# Autodesk Inventor assembly: Leg_joint_roll_pitch
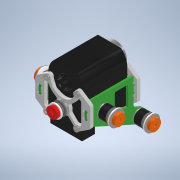
[picture p0: Inventor's stored thumbnail of the model, 180x180]
Saved by Autodesk Inventor 2020 (Build 240168000, 168)
## iProperties
Part Number: Leg_joint_roll_pitch
Document SubType Name: Assembly
Designer: Masato Kubotera
Mass: 101.309 g
Surface Area: 368.925 cm^2
Volume: 74.117 cm^3
Density: 1.36688 g/cm^3
Author: Masato Kubotera
## Documents named in this file (20)
- C:\Users\MasatoKubotera\Documents\Inventor\SUSTAINA-OP\LowerBody\Leg_joit\Leg_joint_roll_pitch.iam
- C:\Users\MasatoKubotera\Documents\Inventor\SUSTAINA-OP\LowerBody\Leg_joit\Leg_joint_pitch_frame.ipt
- C:\Users\MasatoKubotera\Documents\Inventor\SUSTAINA-OP\LowerBody\Leg_joit\Leg_joint_roll_frame.ipt
- C:\Users\MasatoKubotera\Documents\Inventor\SUSTAINA-OP\ReadyMade\Screw\M2_6-20.ipt
- C:\Users\MasatoKubotera\Documents\Inventor\SUSTAINA-OP\ReadyMade\Screw\M2_6-15.ipt
- C:\Users\MasatoKubotera\Documents\Inventor\SUSTAINA-OP\ReadyMade\Bush\80F-0603.ipt
- C:\Users\MasatoKubotera\Documents\Inventor\SUSTAINA-OP\ReadyMade\Washer\CC-0612-50B.ipt
- C:\Users\MasatoKubotera\Documents\Inventor\SUSTAINA-OP\ReadyMade\InsertNut\SF419.ipt
- C:\Users\MasatoKubotera\Documents\Inventor\SUSTAINA-OP\ReadyMade\Washer\UUW-0412-10H.ipt
- C:\Users\MasatoKubotera\Documents\Inventor\SUSTAINA-OP\ReadyMade\Spacer\SLSBF6-39.5-M4-N4.ipt
- C:\Users\MasatoKubotera\Documents\Inventor\SUSTAINA-OP\ReadyMade\Screw\DBTS4-11-6-DHC.ipt
- C:\Users\MasatoKubotera\Documents\Inventor\SUSTAINA-OP\ReadyMade\Screw\DBTS4-5-5-DHC.ipt
- C:\Users\MasatoKubotera\Documents\Inventor\SUSTAINA-OP\ReadyMade\Screw\DBTS4-10-4-DHC.ipt
- C:\Users\MasatoKubotera\Documents\Inventor\SUSTAINA-OP\ReadyMade\InsertNut\S4-05-3W.ipt
- C:\Users\MasatoKubotera\Documents\Inventor\SUSTAINA-OP\ReadyMade\Screw\DBTS4-11-8-DHC.ipt
- C:\Users\MasatoKubotera\Documents\Inventor\SUSTAINA-OP\ReadyMade\Washer\UUW-0614-05H.ipt
- C:\Users\MasatoKubotera\Documents\Inventor\SUSTAINA-OP\ReadyMade\Washer\TT-0612-10.ipt
- C:\Users\MasatoKubotera\Documents\Inventor\SUSTAINA-OP\ReadyMade\Washer\TT-0814-10.ipt
- C:\Users\MasatoKubotera\Documents\Inventor\SUSTAINA-OP\ReadyMade\Washer\CCC-0612-65B.ipt
- C:\Users\MasatoKubotera\Documents\Inventor\SUSTAINA-OP\ReadyMade\KONDO\B3M-SC-1170-A_with_ClampHorn.iam
## Components (50 placed, 19 different names)
1. Leg_joint_roll_frame:1 — 挿入:5, 挿入:6, 挿入:7, 挿入:8, 挿入:9, 挿入:10, 角度:1, フラッシュ:2, メイト:3, メイト:4, メイト:5, 挿入:248, 挿入:249
2. Leg_joint_roll_frame:2 — 挿入:15, 挿入:16, 挿入:17, 挿入:18, 角度:2, 角度:4, 挿入:246, 挿入:247
3. Leg_joint_pitch_frame:1 — フラッシュ:3, 挿入:19, フラッシュ:4, メイト:5, 挿入:20, 挿入:21, 挿入:22
4. Leg_joint_pitch_frame:2 — フラッシュ:2, フラッシュ:3, フラッシュ:4, メイト:3, メイト:4, 挿入:23, 挿入:24, 挿入:25, 挿入:26
5. 80F-0603:1 — 挿入:43
6. 80F-0603:2 — 挿入:44
7. 80F-0603:3 — 挿入:243
8. 80F-0603:4 — 挿入:242
9. 80F-0603:5 — 挿入:244
10. 80F-0603:6 — 挿入:245
11. UUW-0412-10BH:1 — 挿入:9, 挿入:27
12. UUW-0412-10BH:2 — 挿入:17, 挿入:28, 挿入:33
13. UUW-0412-10BH:3 — 挿入:19, 挿入:226, 挿入:241
14. UUW-0412-10BH:4 — 挿入:22, 挿入:35, 挿入:240
15. UUW-0412-10BH:5 — 挿入:23, 挿入:227, 挿入:239
16. UUW-0412-10BH:6 — 挿入:26, 挿入:37, 挿入:238
17. UUW-0412-10BH:7 — 挿入:27, 挿入:38, 挿入:43
18. CC-0612-50B:5 — 挿入:28, 挿入:44
19. SF419:1 — 挿入:25
20. SF419:2 — 挿入:20
21. S4-05-3W:1 — 挿入:10, 角度:1
22. S4-05-3W:2 — 挿入:18, 角度:2
23. SLSBF6-39.5-M4-N4:1 — 挿入:21, 挿入:24, 角度:4
24. DBS4-5-5:1 — 挿入:38, 挿入:232
25. DBTS4-11-6:3 — 挿入:37, 挿入:229
26. DBTS4-11-6:4 — 挿入:35, 挿入:230
27. DBTS4-10-4:1 — 挿入:33, 挿入:233
28. DBTS4-11-8:1 — 挿入:226, 挿入:231
29. DBTS4-11-8:2 — 挿入:227, 挿入:228
30. UUW-0614-05BH:1 — 挿入:228, 挿入:234
31. UUW-0614-05BH:2 — 挿入:229, 挿入:235
32. UUW-0614-05BH:3 — 挿入:230, 挿入:236
33. UUW-0614-05BH:4 — 挿入:231, 挿入:237
34. TT-0612-10:1 — 挿入:233
35. TT-0612-10:2 — 挿入:232
36. TT-0814-10:1 — 挿入:234
37. TT-0814-10:2 — 挿入:235
38. TT-0814-10:3 — 挿入:237
39. TT-0814-10:4 — 挿入:236
40. CCC-0612-65B:1 — 挿入:238, 挿入:245
41. CCC-0612-65B:2 — 挿入:241, 挿入:243
42. CCC-0612-65B:3 — 挿入:239, 挿入:244
43. CCC-0612-65B:4 — 挿入:240, 挿入:242
44. B3M-SC-1170-A_with_ClampHorn:1 [sub-assembly] — 挿入:246, 挿入:247, 挿入:248, 挿入:249
45. M2_6-20:1 — 挿入:7
46. M2_6-20:2 — 挿入:8
47. M2_6-20:3 — 挿入:5
48. M2_6-20:4 — 挿入:6
49. M2_6-15:2 — 挿入:16
50. M2_6-15:3 — 挿入:15
## Relationships (59: Insert 50, Angle 3, Flush 3, Mate 3)
- 挿入:5 [Insert]: Leg_joint_roll_frame:1 ↔ M2_6-20:3
- 挿入:6 [Insert]: Leg_joint_roll_frame:1 ↔ M2_6-20:4
- 挿入:7 [Insert]: Leg_joint_roll_frame:1 ↔ M2_6-20:1
- 挿入:8 [Insert]: Leg_joint_roll_frame:1 ↔ M2_6-20:2
- 挿入:9 [Insert]: Leg_joint_roll_frame:1 ↔ UUW-0412-10BH:1
- 挿入:10 [Insert]: Leg_joint_roll_frame:1 ↔ S4-05-3W:1
- 角度:1 [Angle] (0 deg): Leg_joint_roll_frame:1 ↔ S4-05-3W:1
- 挿入:15 [Insert]: Leg_joint_roll_frame:2 ↔ M2_6-15:3
- 挿入:16 [Insert]: Leg_joint_roll_frame:2 ↔ M2_6-15:2
- 挿入:17 [Insert]: Leg_joint_roll_frame:2 ↔ UUW-0412-10BH:2
- 挿入:18 [Insert]: Leg_joint_roll_frame:2 ↔ S4-05-3W:2
- 角度:2 [Angle] (0 deg): Leg_joint_roll_frame:2 ↔ S4-05-3W:2
- 挿入:19 [Insert]: Leg_joint_pitch_frame:1 ↔ UUW-0412-10BH:3
- 挿入:20 [Insert]: Leg_joint_pitch_frame:1 ↔ SF419:2
- 挿入:21 [Insert]: Leg_joint_pitch_frame:1 ↔ SLSBF6-39.5-M4-N4:1
- 挿入:22 [Insert]: Leg_joint_pitch_frame:1 ↔ UUW-0412-10BH:4
- 挿入:23 [Insert]: Leg_joint_pitch_frame:2 ↔ UUW-0412-10BH:5
- 挿入:24 [Insert]: Leg_joint_pitch_frame:2 ↔ SLSBF6-39.5-M4-N4:1
- 挿入:25 [Insert]: Leg_joint_pitch_frame:2 ↔ SF419:1
- 挿入:26 [Insert]: Leg_joint_pitch_frame:2 ↔ UUW-0412-10BH:6
- 挿入:27 [Insert]: UUW-0412-10BH:1 ↔ UUW-0412-10BH:7
- 挿入:28 [Insert]: UUW-0412-10BH:2 ↔ CC-0612-50B:5
- 挿入:33 [Insert]: UUW-0412-10BH:2 ↔ DBTS4-10-4:1
- 挿入:35 [Insert]: UUW-0412-10BH:4 ↔ DBTS4-11-6:4
- 挿入:37 [Insert]: UUW-0412-10BH:6 ↔ DBTS4-11-6:3
- 挿入:38 [Insert]: UUW-0412-10BH:7 ↔ DBS4-5-5:1
- 挿入:43 [Insert]: 80F-0603:1 ↔ UUW-0412-10BH:7
- 挿入:44 [Insert]: 80F-0603:2 ↔ CC-0612-50B:5
- フラッシュ:2 [Flush]: Leg_joint_roll_frame:1 ↔ Leg_joint_pitch_frame:2
- フラッシュ:3 [Flush]: Leg_joint_pitch_frame:1 ↔ Leg_joint_pitch_frame:2
- フラッシュ:4 [Flush]: Leg_joint_pitch_frame:1 ↔ Leg_joint_pitch_frame:2
- メイト:3 [Mate] (0.025 mm): Leg_joint_roll_frame:1 ↔ Leg_joint_pitch_frame:2
- メイト:4 [Mate] (0.025 mm): Leg_joint_roll_frame:1 ↔ Leg_joint_pitch_frame:2
- メイト:5 [Mate] (0.025 mm): Leg_joint_roll_frame:1 ↔ Leg_joint_pitch_frame:1
- 角度:4 [Angle] (0 deg): Leg_joint_roll_frame:2 ↔ SLSBF6-39.5-M4-N4:1
- 挿入:226 [Insert]: UUW-0412-10BH:3 ↔ DBTS4-11-8:1
- 挿入:227 [Insert]: UUW-0412-10BH:5 ↔ DBTS4-11-8:2
- 挿入:228 [Insert]: DBTS4-11-8:2 ↔ UUW-0614-05BH:1
- 挿入:229 [Insert]: DBTS4-11-6:3 ↔ UUW-0614-05BH:2
- 挿入:230 [Insert]: DBTS4-11-6:4 ↔ UUW-0614-05BH:3
- 挿入:231 [Insert]: DBTS4-11-8:1 ↔ UUW-0614-05BH:4
- 挿入:232 [Insert]: DBS4-5-5:1 ↔ TT-0612-10:2
- 挿入:233 [Insert]: DBTS4-10-4:1 ↔ TT-0612-10:1
- 挿入:234 [Insert]: UUW-0614-05BH:1 ↔ TT-0814-10:1
- 挿入:235 [Insert]: UUW-0614-05BH:2 ↔ TT-0814-10:2
- 挿入:236 [Insert]: UUW-0614-05BH:3 ↔ TT-0814-10:4
- 挿入:237 [Insert]: UUW-0614-05BH:4 ↔ TT-0814-10:3
- 挿入:238 [Insert]: UUW-0412-10BH:6 ↔ CCC-0612-65B:1
- 挿入:239 [Insert]: UUW-0412-10BH:5 ↔ CCC-0612-65B:3
- 挿入:240 [Insert]: UUW-0412-10BH:4 ↔ CCC-0612-65B:4
- 挿入:241 [Insert]: UUW-0412-10BH:3 ↔ CCC-0612-65B:2
- 挿入:242 [Insert]: 80F-0603:4 ↔ CCC-0612-65B:4
- 挿入:243 [Insert]: 80F-0603:3 ↔ CCC-0612-65B:2
- 挿入:244 [Insert]: 80F-0603:5 ↔ CCC-0612-65B:3
- 挿入:245 [Insert]: 80F-0603:6 ↔ CCC-0612-65B:1
- 挿入:246 [Insert]: Leg_joint_roll_frame:2 ↔ B3M-SC-1170-A_with_ClampHorn:1
- 挿入:247 [Insert]: Leg_joint_roll_frame:2 ↔ B3M-SC-1170-A_with_ClampHorn:1
- 挿入:248 [Insert]: Leg_joint_roll_frame:1 ↔ B3M-SC-1170-A_with_ClampHorn:1
- 挿入:249 [Insert]: Leg_joint_roll_frame:1 ↔ B3M-SC-1170-A_with_ClampHorn:1
